# Autodesk Inventor assembly: Assembly Plate Assembly
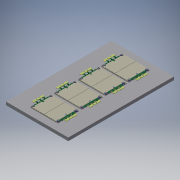
[picture p0: Inventor's stored thumbnail of the model, 180x180]
Saved by Autodesk Inventor 2019.4 (Build 234330000, 330)
## iProperties
Created: 2021-01-11
Part Number: Assembly Plate Assembly
Document SubType Name: Assembly
Designer: caleb
Author: caleb
## Documents named in this file (3)
- C:\Users\cfang\Desktop\nebraska-silicon-lab\CAD\ETL\Module Assembly\Assembly Plate\Assembly Plate Assembly.iam
- C:\Users\cfang\Desktop\nebraska-silicon-lab\CAD\ETL\Module Assembly\Assembly Plate\Assembly Plate.ipt
- C:\Users\cfang\Desktop\nebraska-silicon-lab\CAD\ETL\modules\tdr\F10110887--_1-MODULE_ CMS2 ETL_ FULL DBL-SENSOR MOUNTED ASSY.iam
## Components (5 placed, 2 different names)
1. Assembly Plate:1 — Mate:1, Mate:2, Mate:3, Mate:4, Angle:1, Angle:2, Angle:3, Angle:4
2. F10110887--_1-MODULE_ CMS2 ETL_ FULL DBL-SENSOR MOUNTED ASSY:1 [sub-assembly] — Mate:1, Angle:1, Flush:1, Flush:2, Flush:3
3. F10110887--_1-MODULE_ CMS2 ETL_ FULL DBL-SENSOR MOUNTED ASSY:2 [sub-assembly] — Mate:2, Angle:2, Flush:1
4. F10110887--_1-MODULE_ CMS2 ETL_ FULL DBL-SENSOR MOUNTED ASSY:3 [sub-assembly] — Mate:3, Angle:3, Flush:2
5. F10110887--_1-MODULE_ CMS2 ETL_ FULL DBL-SENSOR MOUNTED ASSY:4 [sub-assembly] — Mate:4, Angle:4, Flush:3
## Relationships (11: Mate 4, Angle 4, Flush 3)
- Mate:1: Assembly Plate:1 ↔ F10110887--_1-MODULE_ CMS2 ETL_ FULL DBL-SENSOR MOUNTED ASSY:1
- Mate:2: Assembly Plate:1 ↔ F10110887--_1-MODULE_ CMS2 ETL_ FULL DBL-SENSOR MOUNTED ASSY:2
- Mate:3: Assembly Plate:1 ↔ F10110887--_1-MODULE_ CMS2 ETL_ FULL DBL-SENSOR MOUNTED ASSY:3
- Mate:4: Assembly Plate:1 ↔ F10110887--_1-MODULE_ CMS2 ETL_ FULL DBL-SENSOR MOUNTED ASSY:4
- Angle:1 (0 deg): Assembly Plate:1 ↔ F10110887--_1-MODULE_ CMS2 ETL_ FULL DBL-SENSOR MOUNTED ASSY:1
- Angle:2 (0 deg): Assembly Plate:1 ↔ F10110887--_1-MODULE_ CMS2 ETL_ FULL DBL-SENSOR MOUNTED ASSY:2
- Angle:3 (0 deg): Assembly Plate:1 ↔ F10110887--_1-MODULE_ CMS2 ETL_ FULL DBL-SENSOR MOUNTED ASSY:3
- Angle:4 (0 deg): Assembly Plate:1 ↔ F10110887--_1-MODULE_ CMS2 ETL_ FULL DBL-SENSOR MOUNTED ASSY:4
- Flush:1: F10110887--_1-MODULE_ CMS2 ETL_ FULL DBL-SENSOR MOUNTED ASSY:1 ↔ F10110887--_1-MODULE_ CMS2 ETL_ FULL DBL-SENSOR MOUNTED ASSY:2
- Flush:2: F10110887--_1-MODULE_ CMS2 ETL_ FULL DBL-SENSOR MOUNTED ASSY:1 ↔ F10110887--_1-MODULE_ CMS2 ETL_ FULL DBL-SENSOR MOUNTED ASSY:3
- Flush:3: F10110887--_1-MODULE_ CMS2 ETL_ FULL DBL-SENSOR MOUNTED ASSY:1 ↔ F10110887--_1-MODULE_ CMS2 ETL_ FULL DBL-SENSOR MOUNTED ASSY:4
